# Autodesk Inventor assembly: DetektorElektronik_Stage1
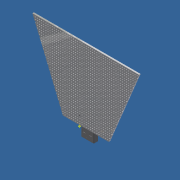
[picture p0: Inventor's stored thumbnail of the model, 180x180]
Saved by Autodesk Inventor 2018 (Build 220112000, 112)
## iProperties
Created: 2018-11-01
Part Number: DetektorElektronik_Stage1
Material: Generisch
Document SubType Name: Assembly
Designer: M.Knabel
Author: M.Knabel
## Documents named in this file (5)
- C:\Users\knabe\Documents\Nicole\Uni\COSIMA\CAD\Detektormodul\DetektorElektronik_Stage1.iam
- C:\Users\knabe\Documents\Nicole\Uni\COSIMA\CAD\Detektormodul\Detektorplatine.ipt
- C:\Users\knabe\Documents\Nicole\Uni\COSIMA\CAD\Detektormodul\USB_male.ipt
- C:\Users\knabe\Documents\Nicole\Uni\COSIMA\CAD\Oktokommander\Adafruit.ipt
- C:\Users\knabe\Documents\Nicole\Uni\COSIMA\CAD\Oktokommander\16Bit I2C ADC+PGA - ADS1115.iam
## Components (4 placed, 4 different names)
1. Detektorplatine:1 — Fluchtend:1, Passend:1, Passend:2, Passend:3
2. USB_male:1 — Fluchtend:1, Passend:1, Passend:2
3. Adafruit:1 — Passend:3, Passend:4
4. 16Bit I2C ADC+PGA - ADS1115:1 [sub-assembly] — Passend:4
## Relationships (5: Mate 4, Flush 1)
- Fluchtend:1 [Flush] (-10 mm): Detektorplatine:1 ↔ USB_male:1
- Passend:1 [Mate]: Detektorplatine:1 ↔ USB_male:1
- Passend:2 [Mate] (15.647 mm): Detektorplatine:1 ↔ USB_male:1
- Passend:3 [Mate] (3 mm): Detektorplatine:1 ↔ Adafruit:1
- Passend:4 [Mate]: Adafruit:1 ↔ 16Bit I2C ADC+PGA - ADS1115:1
